# Autodesk Inventor assembly: Assembly3
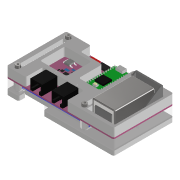
[picture p0: Inventor's stored thumbnail of the model, 180x180]
Saved by Autodesk Inventor 2020 (Build 240168000, 168)
## iProperties
Created: 2021-07-01
Part Number: Assembly3
Document SubType Name: Assembly
Designer: ferrerx
Author: ferrerx
## Documents named in this file (13)
- C:\Users\ferrerx\Documents\GitHub\Sport_Analyzer\Design Files\Mechanical\Assembly3.iam
- C:\Users\ferrerx\Documents\GitHub\Sport_Analyzer\Design Files\Mechanical\Sport Analyzer 1.0.1 PCB .iam
- C:\Users\ferrerx\Documents\GitHub\Sport_Analyzer\Design Files\Mechanical\Bottom PMMA.ipt
- C:\Users\ferrerx\Documents\GitHub\Sport_Analyzer\Design Files\Mechanical\Middle PMMA.ipt
- C:\Users\ferrerx\Documents\GitHub\Sport_Analyzer\Design Files\Mechanical\Top PMMA.ipt
- C:\Users\ferrerx\Documents\GitHub\Sport_Analyzer\Design Files\Mechanical\Adafruit 2.8TFT.ipt
- C:\Users\ferrerx\Documents\GitHub\Sport_Analyzer\Design Files\Mechanical\RJ12 Connector.ipt
- C:\Users\ferrerx\Documents\GitHub\Sport_Analyzer\Design Files\Mechanical\9V Battery.ipt
- C:\Users\ferrerx\Documents\GitHub\Sport_Analyzer\Design Files\Mechanical\Body_Housing 9V Battery.ipt
- C:\Users\ferrerx\Documents\GitHub\Sport_Analyzer\Design Files\Mechanical\Teensy3.2.ipt
- C:\Users\ferrerx\Documents\GitHub\Sport_Analyzer\Design Files\Mechanical\Sport Analyzer 1.0.1 PCB (2) .ipt
- C:\Users\ferrerx\Documents\Inventor\Content Center Files\R2020\en-US\BS 4168(1)\BS 4168 - M3 x 16(1).ipt
- C:\Users\ferrerx\Documents\GitHub\Sport_Analyzer\Design Files\Mechanical\Spacer.ipt
## Components (23 placed, 12 different names)
1. Sport Analyzer 1.0.1 PCB :1 [sub-assembly] — Mate:1, Flush:1, Flush:2, Mate:2, Flush:7, Mate:3, Mate:4, Mate:10, Mate:11, Mate:12, Mate:15, Mate:16, Mate:17, Flush:9, Flush:10, Mate:18
2. Bottom PMMA:1 — Mate:1, Flush:1, Flush:2, Flush:3, Flush:4, Flush:8, Mate:27, Mate:28, Mate:29, Mate:30, Mate:39, Mate:40, Mate:41, Mate:42
3. Middle PMMA:1 — Flush:3, Mate:2, Flush:4, Flush:5, Flush:6, Mate:5, Angle:1, Mate:13
4. Top PMMA:1 — Flush:5, Flush:6, Mate:19, Mate:20, Mate:21, Mate:22, Mate:35, Mate:36, Mate:37, Mate:38
5. Adafruit 2.8TFT:1 — Mate:5, Angle:1, Mate:13
6. RJ12 Connector:1 — Flush:7, Mate:3
7. RJ12 Connector:2 — Mate:4, Flush:8
8. 9V Battery:1 — Mate:7, Mate:8, Mate:9
9. Body_Housing 9V Battery:1 — Mate:7, Mate:8, Mate:9, Mate:10, Mate:11, Mate:12
10. Teensy3.2:1 — Mate:15, Mate:16, Mate:17
11. Sport Analyzer 1.0.1 PCB (2) :1 — Flush:9, Flush:10, Mate:18, Mate:31, Mate:32, Mate:33, Mate:34
12. BS 4168 : Part 1 Hexagon Socket Head Cap Screw - Metric M3 x 16:1 — Mate:30, Mate:42
13. BS 4168 : Part 1 Hexagon Socket Head Cap Screw - Metric M3 x 16:2 — Mate:29, Mate:41
14. BS 4168 : Part 1 Hexagon Socket Head Cap Screw - Metric M3 x 16:3 — Mate:28, Mate:40
15. BS 4168 : Part 1 Hexagon Socket Head Cap Screw - Metric M3 x 16:4 — Mate:27, Mate:39
16. BS 4168 : Part 1 Hexagon Socket Head Cap Screw - Metric M3 x 16:5 — Mate:26, Mate:35
17. BS 4168 : Part 1 Hexagon Socket Head Cap Screw - Metric M3 x 16:6 — Mate:25, Mate:38
18. BS 4168 : Part 1 Hexagon Socket Head Cap Screw - Metric M3 x 16:7 — Mate:23, Mate:37
19. BS 4168 : Part 1 Hexagon Socket Head Cap Screw - Metric M3 x 16:8 — Mate:24, Mate:36
20. Spacer:1 — Mate:19, Mate:25, Mate:32
21. Spacer:2 — Mate:20, Mate:26, Mate:31
22. Spacer:3 — Mate:22, Mate:24, Mate:33
23. Spacer:4 — Mate:21, Mate:23, Mate:34
## Relationships (51: Mate 40, Flush 10, Angle 1)
- Mate:1: Sport Analyzer 1.0.1 PCB :1 ↔ Bottom PMMA:1
- Flush:1: Sport Analyzer 1.0.1 PCB :1 ↔ Bottom PMMA:1
- Flush:2: Sport Analyzer 1.0.1 PCB :1 ↔ Bottom PMMA:1
- Flush:3: Bottom PMMA:1 ↔ Middle PMMA:1
- Mate:2: Sport Analyzer 1.0.1 PCB :1 ↔ Middle PMMA:1
- Flush:4: Bottom PMMA:1 ↔ Middle PMMA:1
- Flush:5: Middle PMMA:1 ↔ Top PMMA:1
- Flush:6: Middle PMMA:1 ↔ Top PMMA:1
- Flush:7: Sport Analyzer 1.0.1 PCB :1 ↔ RJ12 Connector:1
- Mate:3: Sport Analyzer 1.0.1 PCB :1 ↔ RJ12 Connector:1
- Mate:4: Sport Analyzer 1.0.1 PCB :1 ↔ RJ12 Connector:2
- Flush:8: Bottom PMMA:1 ↔ RJ12 Connector:2
- Mate:5: Middle PMMA:1 ↔ Adafruit 2.8TFT:1
- Angle:1 (0 deg): Middle PMMA:1 ↔ Adafruit 2.8TFT:1
- Mate:7: 9V Battery:1 ↔ Body_Housing 9V Battery:1
- Mate:8: 9V Battery:1 ↔ Body_Housing 9V Battery:1
- Mate:9 (1 mm): 9V Battery:1 ↔ Body_Housing 9V Battery:1
- Mate:10: Sport Analyzer 1.0.1 PCB :1 ↔ Body_Housing 9V Battery:1
- Mate:11: Sport Analyzer 1.0.1 PCB :1 ↔ Body_Housing 9V Battery:1
- Mate:12: Sport Analyzer 1.0.1 PCB :1 ↔ Body_Housing 9V Battery:1
- Mate:13: Middle PMMA:1 ↔ Adafruit 2.8TFT:1
- Mate:15: Sport Analyzer 1.0.1 PCB :1 ↔ Teensy3.2:1
- Mate:16: Sport Analyzer 1.0.1 PCB :1 ↔ Teensy3.2:1
- Mate:17: Sport Analyzer 1.0.1 PCB :1 ↔ Teensy3.2:1
- Flush:9: Sport Analyzer 1.0.1 PCB :1 ↔ Sport Analyzer 1.0.1 PCB (2) :1
- Flush:10: Sport Analyzer 1.0.1 PCB :1 ↔ Sport Analyzer 1.0.1 PCB (2) :1
- Mate:18: Sport Analyzer 1.0.1 PCB :1 ↔ Sport Analyzer 1.0.1 PCB (2) :1
- Mate:19: Top PMMA:1 ↔ Spacer:1
- Mate:20: Top PMMA:1 ↔ Spacer:2
- Mate:21: Top PMMA:1 ↔ Spacer:4
- Mate:22: Top PMMA:1 ↔ Spacer:3
- Mate:23: BS 4168 : Part 1 Hexagon Socket Head Cap Screw - Metric M3 x 16:7 ↔ Spacer:4
- Mate:24: BS 4168 : Part 1 Hexagon Socket Head Cap Screw - Metric M3 x 16:8 ↔ Spacer:3
- Mate:25: BS 4168 : Part 1 Hexagon Socket Head Cap Screw - Metric M3 x 16:6 ↔ Spacer:1
- Mate:26: BS 4168 : Part 1 Hexagon Socket Head Cap Screw - Metric M3 x 16:5 ↔ Spacer:2
- Mate:27: Bottom PMMA:1 ↔ BS 4168 : Part 1 Hexagon Socket Head Cap Screw - Metric M3 x 16:4
- Mate:28: Bottom PMMA:1 ↔ BS 4168 : Part 1 Hexagon Socket Head Cap Screw - Metric M3 x 16:3
- Mate:29: Bottom PMMA:1 ↔ BS 4168 : Part 1 Hexagon Socket Head Cap Screw - Metric M3 x 16:2
- Mate:30: Bottom PMMA:1 ↔ BS 4168 : Part 1 Hexagon Socket Head Cap Screw - Metric M3 x 16:1
- Mate:31: Sport Analyzer 1.0.1 PCB (2) :1 ↔ Spacer:2
- Mate:32: Sport Analyzer 1.0.1 PCB (2) :1 ↔ Spacer:1
- Mate:33: Sport Analyzer 1.0.1 PCB (2) :1 ↔ Spacer:3
- Mate:34: Sport Analyzer 1.0.1 PCB (2) :1 ↔ Spacer:4
- Mate:35: Top PMMA:1 ↔ BS 4168 : Part 1 Hexagon Socket Head Cap Screw - Metric M3 x 16:5
- Mate:36: Top PMMA:1 ↔ BS 4168 : Part 1 Hexagon Socket Head Cap Screw - Metric M3 x 16:8
- Mate:37: Top PMMA:1 ↔ BS 4168 : Part 1 Hexagon Socket Head Cap Screw - Metric M3 x 16:7
- Mate:38: Top PMMA:1 ↔ BS 4168 : Part 1 Hexagon Socket Head Cap Screw - Metric M3 x 16:6
- Mate:39: Bottom PMMA:1 ↔ BS 4168 : Part 1 Hexagon Socket Head Cap Screw - Metric M3 x 16:4
- Mate:40: Bottom PMMA:1 ↔ BS 4168 : Part 1 Hexagon Socket Head Cap Screw - Metric M3 x 16:3
- Mate:41: Bottom PMMA:1 ↔ BS 4168 : Part 1 Hexagon Socket Head Cap Screw - Metric M3 x 16:2
- Mate:42: Bottom PMMA:1 ↔ BS 4168 : Part 1 Hexagon Socket Head Cap Screw - Metric M3 x 16:1
